# Autodesk Inventor assembly: Motor+BottomToBottom
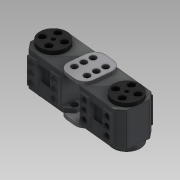
[picture p0: Inventor's stored thumbnail of the model, 180x180]
Saved by Autodesk Inventor 2014 (Build 180170000, 170)
## iProperties
Created: 2014-03-07
Part Number: Motor+BottomToBottom
Document SubType Name: Assembly
Designer: Grégoire
Author: Grégoire
## Documents named in this file (5)
- C:\Users\Grégoire\Desktop\XL320\src\Motor+BottomToBottom.iam
- C:\Users\Grégoire\Desktop\XL320\src\Motor.ipt
- C:\Users\Grégoire\Desktop\XL320\src\Arm.ipt
- C:\Users\Grégoire\Desktop\XL320\src\CounterArm.ipt
- C:\Users\Grégoire\Desktop\XL320\src\BottomToBottom.ipt
## Components (8 placed, 4 different names)
1. Motor:1 — Placage:1, Placage:2, Placage:3, Placage:4, Placage:9, Placage:10, Placage:11, Placage:12, Placage:13, Placage:14
2. Arm:1 — Placage:3, Placage:4
3. CounterArm:1 — Placage:1, Placage:2
4. Motor:2 — Placage:15, Placage:16, Placage:17
5. Arm:2
6. CounterArm:2
7. BottomToBottom:1 — Placage:9, Placage:10, Placage:11
8. BottomToBottom:2 — Placage:12, Placage:13, Placage:14, Placage:15, Placage:16, Placage:17
## Relationships (17: Mate 17)
- Placage:1 [Mate]: Motor:1 ↔ CounterArm:1
- Placage:2 [Mate]: Motor:1 ↔ CounterArm:1
- Placage:3 [Mate]: Motor:1 ↔ Arm:1
- Placage:4 [Mate]: Motor:1 ↔ Arm:1
- [Mate]: Motor:2 ↔ CounterArm:2
- [Mate]: Motor:2 ↔ CounterArm:2
- [Mate]: Motor:2 ↔ Arm:2
- [Mate]: Motor:2 ↔ Arm:2
- Placage:9 [Mate]: Motor:1 ↔ BottomToBottom:1
- Placage:10 [Mate]: Motor:1 ↔ BottomToBottom:1
- Placage:11 [Mate]: Motor:1 ↔ BottomToBottom:1
- Placage:12 [Mate]: Motor:1 ↔ BottomToBottom:2
- Placage:13 [Mate]: Motor:1 ↔ BottomToBottom:2
- Placage:14 [Mate]: Motor:1 ↔ BottomToBottom:2
- Placage:15 [Mate]: Motor:2 ↔ BottomToBottom:2
- Placage:16 [Mate]: Motor:2 ↔ BottomToBottom:2
- Placage:17 [Mate]: Motor:2 ↔ BottomToBottom:2
## Named parameters: d20_d0 = 0 mm, d21_d1 = 0 mm, d22_d2 = 0 mm, d23_d3 = 0 mm
